# Autodesk Inventor assembly: panel assembly
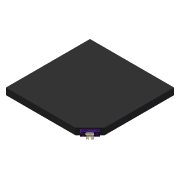
[picture p0: Inventor's stored thumbnail of the model, 180x180]
Saved by Autodesk Inventor 2017 (Build 210142000, 142)
## iProperties
Created: 2016-08-11
Part Number: panel assembly
Document SubType Name: Assembly
Designer: Jonathan
Author: Jonathan
## Documents named in this file (4)
- C:\Users\sawaiz\oneDrive\projects\muonTelescope\panel assembly\panel assembly.iam
- C:\Users\sawaiz\oneDrive\projects\muonTelescope\panel assembly\4-40 half inch screw.ipt
- C:\Users\sawaiz\oneDrive\projects\muonTelescope\dependency\scintilatorPanel\scintillatorPanel.iam
- C:\Users\sawaiz\oneDrive\projects\muonTelescope\dependency\mppcSensor\cad\mppcSensor.iam
## Components (4 placed, 3 different names)
1. 4-40 half inch screw:1 — Mate:3, Flush:1, Mate:5
2. 4-40 half inch screw:2 — Mate:4, Flush:1
3. scintillatorPanel:1 [sub-assembly] — Mate:1, Angle:1, Mate:2
4. mppcSensor:1 [sub-assembly] — Mate:1, Angle:1, Mate:2, Mate:3, Mate:4, Mate:5
## Relationships (7: Mate 5, Angle 1, Flush 1)
- Mate:1: scintillatorPanel:1 ↔ mppcSensor:1
- Angle:1 (0 deg): scintillatorPanel:1 ↔ mppcSensor:1
- Mate:2: scintillatorPanel:1 ↔ mppcSensor:1
- Mate:3: 4-40 half inch screw:1 ↔ mppcSensor:1
- Mate:4: 4-40 half inch screw:2 ↔ mppcSensor:1
- Flush:1: 4-40 half inch screw:1 ↔ 4-40 half inch screw:2
- Mate:5: 4-40 half inch screw:1 ↔ mppcSensor:1
